# Autodesk Inventor assembly: Baugruppe1
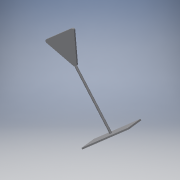
[picture p0: Inventor's stored thumbnail of the model, 180x180]
Saved by Autodesk Inventor 2019.5 (Build 235369000, 369)
## iProperties
Created: 2021-10-06
Part Number: Baugruppe1
Material: Generisch
Document SubType Name: Assembly
Designer: mritt
Author: mritt
## Documents named in this file (3)
- D:\Studium\Universität Stuttgart\Sonstige Tätigkeiten\Tätigkeit_studentische_Hilfskraft_Informatik\Hiwi-Projekt\CAD-Dateien\Arena\Arena Komplettset\Vorfahrtsschild\Baugruppe1.iam
- D:\Studium\Universität Stuttgart\Sonstige Tätigkeiten\Tätigkeit_studentische_Hilfskraft_Informatik\Hiwi-Projekt\CAD-Dateien\Arena\Arena Komplettset\Vorfahrtsschild\Vorfahrtsschild_Teil_Oben.ipt
- D:\Studium\Universität Stuttgart\Sonstige Tätigkeiten\Tätigkeit_studentische_Hilfskraft_Informatik\Hiwi-Projekt\CAD-Dateien\Arena\Arena Komplettset\Vorfahrtsschild\Vorfahrtsschild_Teil_Unten.ipt
## Components (2 placed, 2 different names)
1. Vorfahrtsschild_Teil_Oben:1 — Passend:1
2. Vorfahrtsschild_Teil_Unten:1 — Passend:1
## Relationships (1: Mate 1)
- Passend:1 [Mate] (-130 mm): Vorfahrtsschild_Teil_Oben:1 ↔ Vorfahrtsschild_Teil_Unten:1
